# Autodesk Inventor assembly: Конструкция
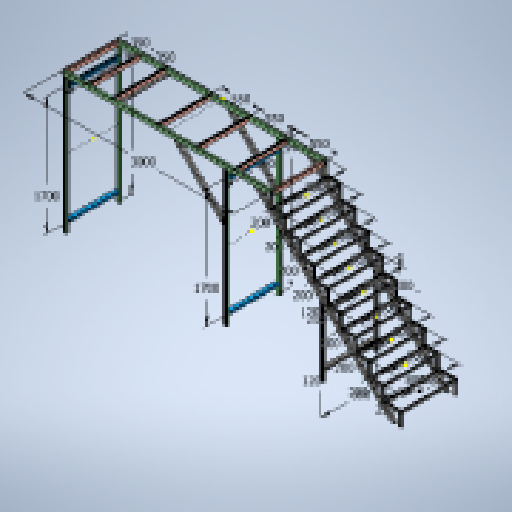
[picture p0: Inventor's stored thumbnail of the model, 512x512]
Saved by Autodesk Inventor 2025 (Build 290162010, 162A)
## iProperties
Created: 2024-08-28
Part Number: Конструкция
Document SubType Name: Assembly
Designer: pokla
Author: pokla
## Documents named in this file (9)
- C:\Users\admin\YandexDisk-badmisterfox\домашниий пк\Inventor\BSH_Beshkino_bio_tank\Конструкция.iam
- C:\Users\admin\YandexDisk-badmisterfox\домашниий пк\Inventor\BSH_Beshkino_bio_tank\лестница\Перегородка\ASY NDM 11.030 перегородка рама 2 горизонт.iam
- C:\Users\admin\YandexDisk-badmisterfox\домашниий пк\Inventor\BSH_Beshkino_bio_tank\лестница\Перегородка\ASY NDM 11.050 перегородка рама 2 вертикал.iam
- C:\Users\admin\YandexDisk-badmisterfox\домашниий пк\Inventor\BSH_Beshkino_bio_tank\Assembly5.iam
- C:\Users\admin\YandexDisk-badmisterfox\домашниий пк\Inventor\BSH_Beshkino_bio_tank\ISO 4019 - 40x20x2 - 180.ipt
- C:\Users\admin\YandexDisk-badmisterfox\домашниий пк\Inventor\BSH_Beshkino_bio_tank\Последняя ступенька.iam
- C:\Users\admin\YandexDisk-badmisterfox\домашниий пк\Inventor\BSH_Beshkino_bio_tank\ISO 4019 - 60x40x3 - 3000.ipt
- C:\Users\admin\YandexDisk-badmisterfox\домашниий пк\Inventor\BSH_Beshkino_bio_tank\ASY NDM рама под лестницей.iam
- C:\Users\admin\YandexDisk-badmisterfox\домашниий пк\Inventor\BSH_Beshkino_bio_tank\ISO 4019 - 60x40x3 - 1000.ipt
## Components (20 placed, 8 different names)
1. ASY NDM 11.030 перегородка рама 2 горизонт:1 [sub-assembly] — Flush:2, Mate:9, Flush:9, Flush:10, Mate:15, Flush:17, Mate:17, Flush:18, Mate:20, Flush:19, Mate:21, Mate:22
2. ASY NDM 11.050 перегородка рама 2 вертикал:1 [sub-assembly] — Mate:9, Flush:9, Flush:10, Flush:15, Mate:16, Mate:18
3. ASY NDM 11.050 перегородка рама 2 вертикал:3 [sub-assembly] — Mate:19
4. Assembly5:1 [sub-assembly] — Flush:2, Rigid:3, Rigid:10, Rigid:11
5. Assembly5:2 [sub-assembly] — Rigid:3, Rigid:4
6. Assembly5:3 [sub-assembly] — Rigid:4, Rigid:5
7. Assembly5:4 [sub-assembly] — Rigid:5, Rigid:6
8. Assembly5:5 [sub-assembly] — Rigid:6, Rigid:7
9. Assembly5:6 [sub-assembly] — Rigid:7, Rigid:8
10. Assembly5:7 [sub-assembly] — Rigid:8, Rigid:9
11. Assembly5:8 [sub-assembly] — Rigid:9, Rigid:12
12. ISO 4019 - 40x20x2 - 180:1 — Rigid:10, Mate:10, Flush:14
13. ISO 4019 - 40x20x2 - 180:2 — Rigid:11, Mate:11, Flush:13
14. Последняя ступенька:1 [sub-assembly] — Rigid:12
15. ISO 4019 - 60x40x3 - 3000:1 — Mate:10, Flush:14, Flush:16, Mate:14, Mate:21
16. ISO 4019 - 60x40x3 - 3000:2 — Mate:11, Flush:13, Mate:22
17. ASY NDM рама под лестницей:1 [sub-assembly] — Flush:15, Flush:16, Mate:14
18. ISO 4019 - 60x40x3 - 1000:1 — Mate:15, Mate:16, Flush:17
19. ISO 4019 - 60x40x3 - 1000:2 — Mate:17, Mate:18, Flush:18
20. ISO 4019 - 60x40x3 - 1000:3 — Mate:19, Mate:20, Flush:19
## Relationships (35: Mate 13, WeldJoint 11, Flush 11)
- [WeldJoint]: ASY NDM 11.030 перегородка рама 2 горизонт:1 ↔ ASY NDM 11.050 перегородка рама 2 вертикал:3
- [Flush]: ASY NDM 11.030 перегородка рама 2 горизонт:1 ↔ Assembly5:1
- [Mate]: ASY NDM 11.030 перегородка рама 2 горизонт:1 ↔ Assembly5:1
- Flush:2 (200 mm): ASY NDM 11.030 перегородка рама 2 горизонт:1 ↔ Assembly5:1
- Mate:9: ASY NDM 11.030 перегородка рама 2 горизонт:1 ↔ ASY NDM 11.050 перегородка рама 2 вертикал:1
- Flush:9: ASY NDM 11.030 перегородка рама 2 горизонт:1 ↔ ASY NDM 11.050 перегородка рама 2 вертикал:1
- Flush:10 (650 mm): ASY NDM 11.030 перегородка рама 2 горизонт:1 ↔ ASY NDM 11.050 перегородка рама 2 вертикал:1
- Rigid:3 [WeldJoint]: Assembly5:1 ↔ Assembly5:2
- Rigid:4 [WeldJoint]: Assembly5:2 ↔ Assembly5:3
- Rigid:5 [WeldJoint]: Assembly5:3 ↔ Assembly5:4
- Rigid:6 [WeldJoint]: Assembly5:4 ↔ Assembly5:5
- Rigid:7 [WeldJoint]: Assembly5:5 ↔ Assembly5:6
- Rigid:8 [WeldJoint]: Assembly5:6 ↔ Assembly5:7
- Rigid:9 [WeldJoint]: Assembly5:7 ↔ Assembly5:8
- Rigid:10 [WeldJoint]: Assembly5:1 ↔ ISO 4019 - 40x20x2 - 180:1
- Rigid:11 [WeldJoint]: Assembly5:1 ↔ ISO 4019 - 40x20x2 - 180:2
- Rigid:12 [WeldJoint]: Assembly5:8 ↔ Последняя ступенька:1
- Mate:10: ISO 4019 - 40x20x2 - 180:1 ↔ ISO 4019 - 60x40x3 - 3000:1
- Mate:11: ISO 4019 - 40x20x2 - 180:2 ↔ ISO 4019 - 60x40x3 - 3000:2
- Flush:13: ISO 4019 - 40x20x2 - 180:2 ↔ ISO 4019 - 60x40x3 - 3000:2
- Flush:14: ISO 4019 - 40x20x2 - 180:1 ↔ ISO 4019 - 60x40x3 - 3000:1
- Flush:15: ASY NDM 11.050 перегородка рама 2 вертикал:1 ↔ ASY NDM рама под лестницей:1
- Flush:16: ISO 4019 - 60x40x3 - 3000:1 ↔ ASY NDM рама под лестницей:1
- Mate:14: ISO 4019 - 60x40x3 - 3000:1 ↔ ASY NDM рама под лестницей:1
- Mate:15: ASY NDM 11.030 перегородка рама 2 горизонт:1 ↔ ISO 4019 - 60x40x3 - 1000:1
- Mate:16: ASY NDM 11.050 перегородка рама 2 вертикал:1 ↔ ISO 4019 - 60x40x3 - 1000:1
- Flush:17: ASY NDM 11.030 перегородка рама 2 горизонт:1 ↔ ISO 4019 - 60x40x3 - 1000:1
- Mate:17: ASY NDM 11.030 перегородка рама 2 горизонт:1 ↔ ISO 4019 - 60x40x3 - 1000:2
- Mate:18: ASY NDM 11.050 перегородка рама 2 вертикал:1 ↔ ISO 4019 - 60x40x3 - 1000:2
- Flush:18: ASY NDM 11.030 перегородка рама 2 горизонт:1 ↔ ISO 4019 - 60x40x3 - 1000:2
- Mate:19: ASY NDM 11.050 перегородка рама 2 вертикал:3 ↔ ISO 4019 - 60x40x3 - 1000:3
- Mate:20: ASY NDM 11.030 перегородка рама 2 горизонт:1 ↔ ISO 4019 - 60x40x3 - 1000:3
- Flush:19: ASY NDM 11.030 перегородка рама 2 горизонт:1 ↔ ISO 4019 - 60x40x3 - 1000:3
- Mate:21: ASY NDM 11.030 перегородка рама 2 горизонт:1 ↔ ISO 4019 - 60x40x3 - 3000:1
- Mate:22: ASY NDM 11.030 перегородка рама 2 горизонт:1 ↔ ISO 4019 - 60x40x3 - 3000:2
